# Autodesk Inventor assembly: m500 mount assembly
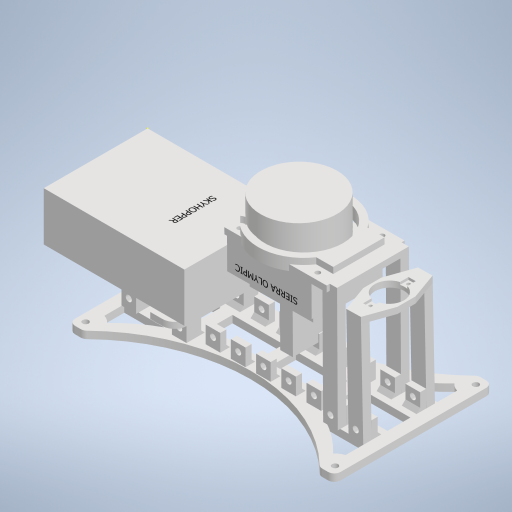
[picture p0: Inventor's stored thumbnail of the model, 512x512]
Saved by Autodesk Inventor 2023 (Build 270158000, 158)
## iProperties
Created: 2022-08-10
Part Number: m500 mount assembly
Document SubType Name: Assembly
Designer: Eli
Author: Eli
## Documents named in this file (7)
- C:\Users\Eli\Documents\inventor parts\m500 mount assembly.iam
- C:\Users\Eli\Documents\inventor parts\m500 mounting plate.ipt
- C:\Users\Eli\Documents\inventor parts\m500 thermal mount.ipt
- C:\Users\Eli\Documents\inventor parts\skyhopper model.ipt
- C:\Users\Eli\Documents\inventor parts\thermal camera model.ipt
- C:\Users\Eli\Documents\inventor parts\m500 skyhopper mount.ipt
- C:\Users\Eli\Documents\inventor parts\m500 hires mount.ipt
## Components (6 placed, 6 different names)
1. m500 mounting plate:1 — Rotational:1, Flush:1, Rotational:4, Rotational:5, Rotational:6, Rotational:7
2. m500 thermal mount:1 — Rotational:1, Mate:2, Flush:1, Rotational:5
3. skyhopper model:1 — Mate:3
4. thermal camera model:1 — Mate:2
5. m500 skyhopper mount:1 — Mate:3, Rotational:6, Rotational:7
6. m500 hires mount:1 — Rotational:4
## Relationships (8: RevoluteJoint 5, Mate 2, Flush 1)
- Rotational:1 [RevoluteJoint]: m500 mounting plate:1 ↔ m500 thermal mount:1
- Mate:2: m500 thermal mount:1 ↔ thermal camera model:1
- Flush:1: m500 mounting plate:1 ↔ m500 thermal mount:1
- Rotational:4 [RevoluteJoint]: m500 mounting plate:1 ↔ m500 hires mount:1
- Rotational:5 [RevoluteJoint]: m500 mounting plate:1 ↔ m500 thermal mount:1
- Mate:3: skyhopper model:1 ↔ m500 skyhopper mount:1
- Rotational:6 [RevoluteJoint]: m500 mounting plate:1 ↔ m500 skyhopper mount:1
- Rotational:7 [RevoluteJoint]: m500 mounting plate:1 ↔ m500 skyhopper mount:1
